# Autodesk Inventor assembly: Assembly1
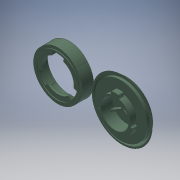
[picture p0: Inventor's stored thumbnail of the model, 180x180]
Saved by Autodesk Inventor 2018 (Build 220112000, 112)
## iProperties
Created: 2020-04-26
Part Number: Assembly1
Document SubType Name: Assembly
Designer: Matt
Author: Matt
## Documents named in this file (4)
- C:\Users\Matt\n95\v5\Assembly1.iam
- C:\Users\Matt\n95\v5\3M  Repirator Adaptors.ipt
- C:\Users\Matt\n95\v5\3MFilterAdapterMaleToolMain.ipt
- C:\Users\Matt\n95\v5\3MFilterAdapterMaleToolMainV2.ipt
## Components (3 placed, 3 different names)
1. 3M  Repirator Adaptors:1 — Flush:1, Flush:2
2. 3MFilterAdapterMaleToolMain:1 — Flush:1
3. 3MFilterAdapterMaleToolMainV2:1 — Flush:2
## Relationships (2: Flush 2)
- Flush:1 (3.175 mm): 3M  Repirator Adaptors:1 ↔ 3MFilterAdapterMaleToolMain:1
- Flush:2: 3M  Repirator Adaptors:1 ↔ 3MFilterAdapterMaleToolMainV2:1
